# Autodesk Inventor assembly: TapeMeasureAssemblyVersion1
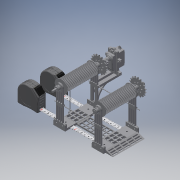
[picture p0: Inventor's stored thumbnail of the model, 180x180]
Saved by Autodesk Inventor 2019 (Build 230136000, 136)
## iProperties
Created: 2018-11-08
Part Number: TapeMeasureAssemblyVersion1
Document SubType Name: Assembly
Designer: Ashley
Author: Ashley
## Documents named in this file (19)
- C:\Users\Ashley\Desktop\repositories\design\inventor\2018-2019\Tape Measure Braket\Version Two\Tape Measure Bracket Assembly V2.iam
- C:\Users\Ashley\Desktop\repositories\design\inventor\2018-2019\Tape Measure Braket\Version Two\Bracket Bottom V2.ipt
- C:\Users\Ashley\Desktop\repositories\design\inventor\2018-2019\Tape Measure Braket\Tape Measure\Tape Measure Edited.iam
- C:\Users\Ashley\Desktop\repositories\design\inventor\2018-2019\Tape Measure Braket\Version Two\Side V2.1.ipt
- C:\Users\Ashley\Desktop\repositories\design\inventor\Imported Components\goBilda\Bearing6mmID.ipt
- C:\Users\Ashley\Desktop\repositories\design\inventor\2018-2019\Tape Measure Braket\Version Three\Pulley Left V3.ipt
- C:\Users\Ashley\Desktop\repositories\design\inventor\Imported Components\goBilda\DShaft140mm.ipt
- C:\Users\Ashley\Desktop\repositories\design\inventor\Imported Components\goBilda\Collar6mm\SetScrewCollar6mmboreassembly.iam
- C:\Users\Ashley\Desktop\repositories\design\inventor\Imported Components\goBilda\DShaft160mm.ipt
- C:\Users\Ashley\Desktop\repositories\design\inventor\2018-2019\Tape Measure Braket\Finished Parts\2mmAxel.ipt
- C:\Users\Ashley\Desktop\repositories\design\inventor\Imported Components\goBilda\CampingHub\ClampingHub assembly.iam
- C:\Users\Ashley\Desktop\repositories\design\inventor\Imported Components\goBilda\8mmPlasticPitchSproket.ipt
- C:\Users\Ashley\Desktop\repositories\design\inventor\Imported Components\goBilda\Servo To Shaft\ServoToShaftCoupler.iam
- C:\Users\Ashley\Desktop\repositories\design\inventor\Imported Components\goBilda\goBildaServo.ipt
- C:\Users\Ashley\Desktop\repositories\design\inventor\Imported Components\goBilda\1802SeriesServoFrame.ipt
- C:\Users\Ashley\Desktop\repositories\design\inventor\2018-2019\Tape Measure Braket\Version Two\Side Servo V2.ipt
- C:\Users\Ashley\Desktop\repositories\design\inventor\2018-2019\Tape Measure Braket\Version Two\Braket Top V2.ipt
- C:\Users\Ashley\Desktop\repositories\design\inventor\2018-2019\Tape Measure Braket\Finished Parts\2mmAxel3in.ipt
- C:\Users\Ashley\Desktop\repositories\design\inventor\2018-2019\Tape Measure Braket\Version Three\Pulley Right V3.ipt
## Components (35 placed, 30 different names)
1. Bracket Bottom — Mate:1, Mate:4, Mate:5, Insert:24
2. Tape Measure Right [sub-assembly]
3. Tape Measure Left [sub-assembly]
4. Back Right Side
5. Front Right Side — Mate:1, Insert:2, Insert:11
6. Front Left Side — Insert:3, Insert:10
7. Back Right Bearing — Insert:17
8. Front Right Bearing — Insert:2
9. Front Left Beaing — Insert:3
10. Front Left BEaring — Insert:23
11. Front Right Collar [sub-assembly]
12. Front Axel — Insert:8, Insert:14, Insert:25
13. Front Left Collar [sub-assembly] — Insert:8
14. Back Left Collar [sub-assembly]
15. Back Right Collar [sub-assembly] — Insert:18
16. Back Axel — Insert:17, Insert:18, Insert:19, Insert:20, Insert:26
17. Left axel — Insert:10
18. Right Axel — Insert:11
19. Front Sproket — Insert:12
20. Front Claming Hub [sub-assembly] — Insert:12, Insert:14
21. Back Sproket
22. Back Clamping Hub [sub-assembly] — Insert:19
23. Servo To Shaft Coupler [sub-assembly] — Insert:20, Insert:21
24. Servo — Insert:21, Mate:3
25. Servo Frame — Mate:3
26. Side Servo V2:1 — Insert:23
27. Braket Top V2:1 — Mate:5
28. Braket Top V2:2 — Mate:4
29. Braket Top V2:3
30. Braket Top V2:4
31. 2mmAxel3in:1 — Insert:24
32. Pulley Right V3:1 — Insert:25, Mate:6
33. Pulley Right V3:2 — Insert:26, Symmetry:1
34. Pulley Left V3:1 — Mate:6
35. Pulley Left V3:2 — Symmetry:1
## Relationships (23: Insert 17, Mate 5, Symmetry 1)
- Mate:1: Bracket Bottom ↔ Front Right Side
- Insert:2: Front Right Side ↔ Front Right Bearing
- Insert:3: Front Left Side ↔ Front Left Beaing
- Insert:8 (14 mm): Front Axel ↔ Front Left Collar
- Insert:10 (-30 mm): Front Left Side ↔ Left axel
- Insert:11 (-30 mm): Front Right Side ↔ Right Axel
- Insert:12 (-1 mm): Front Sproket ↔ Front Claming Hub
- [Insert] (-1 mm): Back Sproket ↔ Back Clamping Hub
- Insert:14 (1 mm): Front Axel ↔ Front Claming Hub
- Insert:17 (20 mm): Back Right Bearing ↔ Back Axel
- Insert:18 (12 mm): Back Right Collar ↔ Back Axel
- Insert:19 (11 mm): Back Axel ↔ Back Clamping Hub
- Insert:20 (-6 mm): Back Axel ↔ Servo To Shaft Coupler
- Insert:21 (-3 mm): Servo To Shaft Coupler ↔ Servo
- Mate:3: Servo ↔ Servo Frame
- Insert:23: Front Left BEaring ↔ Side Servo V2:1
- Mate:4: Bracket Bottom ↔ Braket Top V2:2
- Mate:5: Bracket Bottom ↔ Braket Top V2:1
- Insert:24 (-6.5 mm): Bracket Bottom ↔ 2mmAxel3in:1
- Insert:25 (30 mm): Front Axel ↔ Pulley Right V3:1
- Mate:6: Pulley Right V3:1 ↔ Pulley Left V3:1
- Insert:26 (39 mm): Back Axel ↔ Pulley Right V3:2
- Symmetry:1: Pulley Right V3:2 ↔ Pulley Left V3:2
## Named parameters: d26_d25 = -1 mm
